# Autodesk Inventor assembly: Frame 1647030135921
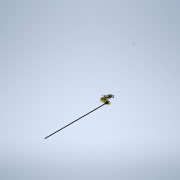
[picture p0: Inventor's stored thumbnail of the model, 180x180]
Saved by Autodesk Inventor 2022.2 (Build 262287000, 287)
## iProperties
_FrameDoc: Frame Assembly
_Version: 25.0.0
Created: 2022-03-11
Part Number: Frame 1647030135921
Document SubType Name: Assembly
Designer: foriw
Mass: 6298.67 g
Surface Area: 9103.39 cm^2
Volume: 2238.81 cm^3
Density: 2.8134 g/cm^3
Author: foriw
## Documents named in this file (31)
- H:\inventor ting\Mekatronik beercart git\Beercart CAD\Workspaces\Workspace\beercart assembly - mekatronik\Frame\Frame 1647030135921.iam
- H:\inventor ting\Mekatronik beercart git\Beercart CAD\Workspaces\Workspace\beercart assembly - mekatronik\Frame\Skeleton 1647030135922.ipt
- H:\inventor ting\Mekatronik beercart git\Beercart CAD\Workspaces\Workspace\beercart assembly - mekatronik\Frame\ISO 12633-2 20x20x2 1647030639616.ipt
- H:\inventor ting\Mekatronik beercart git\Beercart CAD\Workspaces\Workspace\beercart assembly - mekatronik\Frame\ISO 12633-2 20x20x2 1647030639707.ipt
- H:\inventor ting\Mekatronik beercart git\Beercart CAD\Workspaces\Workspace\beercart assembly - mekatronik\Frame\ISO 12633-2 20x20x2 1647606177438.ipt
- H:\inventor ting\Mekatronik beercart git\Beercart CAD\Workspaces\Workspace\BackWheelMountingPlate.ipt
- H:\inventor ting\Mekatronik beercart git\Beercart CAD\Workspaces\Workspace\BackWheelMountingPlate_MIR_MIR.ipt
- H:\inventor ting\Mekatronik beercart git\Beercart CAD\Workspaces\Workspace\bearing housing front.ipt
- H:\inventor ting\Mekatronik beercart git\Beercart CAD\Workspaces\Workspace\beercart assembly - mekatronik\Frame\ISO 12633-2 20x20x2 1648573909221.ipt
- H:\inventor ting\Mekatronik beercart git\Beercart CAD\Workspaces\Workspace\beercart assembly - mekatronik\Frame\ISO 12633-2 20x20x2 1648573975084.ipt
- H:\inventor ting\Mekatronik beercart git\Beercart CAD\Workspaces\Workspace\beercart assembly - mekatronik\Frame\ISO 12633-2 20x20x2 1648627088055.ipt
- H:\inventor ting\Mekatronik beercart git\Beercart CAD\Workspaces\Workspace\beercart assembly - mekatronik\Frame\ISO 12633-2 20x20x2 1648627088175.ipt
- H:\inventor ting\Mekatronik beercart git\Beercart CAD\Workspaces\Workspace\BackWheelMountingPlate_MIR4.ipt
- H:\inventor ting\Mekatronik beercart git\Beercart CAD\Workspaces\Workspace\beercart assembly - mekatronik\Frame\ISO 12633-2 20x20x2 1649085652950.ipt
- H:\inventor ting\Mekatronik beercart git\Beercart CAD\Workspaces\Workspace\beercart assembly - mekatronik\Frame\ISO 12633-2 20x20x2 1649085653040.ipt
- H:\inventor ting\Mekatronik beercart git\Beercart CAD\Workspaces\Workspace\backWheelNoMotor brake mount.ipt
- H:\inventor ting\Mekatronik beercart git\Beercart CAD\Workspaces\Workspace\beercart assembly - mekatronik\Frame\ISO 12633-2 20x20x2 1649154464355.ipt
- H:\inventor ting\Mekatronik beercart git\Beercart CAD\Workspaces\Workspace\BackWheelMotorMountSpacer.ipt
- H:\inventor ting\Mekatronik beercart git\Beercart CAD\Workspaces\Workspace\beercart assembly - mekatronik\Frame\FrontWheelFrameNew.iam
- H:\inventor ting\Mekatronik beercart git\Beercart CAD\Workspaces\Workspace\headset bearing.ipt
- H:\inventor ting\Mekatronik beercart git\Beercart CAD\Workspaces\Workspace\beercart assembly - mekatronik\Frame\ISO 12633-2 20x20x2 1650129877673.ipt
- H:\inventor ting\Mekatronik beercart git\Beercart CAD\Workspaces\Workspace\beercart assembly - mekatronik\Frame\ISO 12633-2 20x20x2 1650129879551.ipt
- H:\inventor ting\Mekatronik beercart git\Beercart CAD\Workspaces\Workspace\beercart assembly - mekatronik\Frame\ISO 12633-2 20x20x2 1650129879650.ipt
- H:\inventor ting\Mekatronik beercart git\Beercart CAD\Workspaces\Workspace\beercart assembly - mekatronik\Frame\ISO 12633-2 20x20x2 1650129879749.ipt
- H:\inventor ting\Mekatronik beercart git\Beercart CAD\Workspaces\Workspace\beercart assembly - mekatronik\Frame\ISO 12633-2 20x20x2 1650134807858.ipt
- H:\inventor ting\Mekatronik beercart git\Beercart CAD\Workspaces\Workspace\bearing housing front_MIR.ipt
- H:\inventor ting\Mekatronik beercart git\Beercart CAD\Libraries\Content Center Files\en-US\ISO 7089\ISO 7089 - 6 - 140 HV(1).ipt
- H:\inventor ting\Mekatronik beercart git\Beercart CAD\Libraries\Content Center Files\en-US\ISO 4762(2)\ISO 4762 - M6 x 16ISO.ipt
- H:\inventor ting\Mekatronik beercart git\Beercart CAD\Workspaces\Workspace\rotating axel.ipt
- H:\inventor ting\Mekatronik beercart git\Beercart CAD\Workspaces\Workspace\beercart assembly - mekatronik\Frame\plan1 .iam
- H:\inventor ting\Mekatronik beercart git\Beercart CAD\Workspaces\Workspace\beercart assembly - mekatronik\Frame\Plan 2 øverste.iam
## Components (36 placed, 26 different names)
1. bearing housing front:1 — Mate:6, Flush:15, Flush:16, Mate:8, Insert:4, Mate:10, Mate:12
2. Reference Skeleton
3. ISO 12633-2 20x20x2 - 250,13:1
4. ISO 12633-2 20x20x2 - 250,13:2
5. ISO 12633-2 20x20x2 - 123,73:2 — Mate:2, Mate:4, Mate:5
6. BackWheelMountingPlate:1 — Flush:6, Rotational:2, Rigid:1
7. BackWheelMountingPlate_MIR_MIR:1
8. ISO 12633-2 20x20x2 - 360,44:1
9. ISO 12633-2 20x20x2 - 105,43:1 — Flush:6, Rotational:2, Rigid:1
10. ISO 12633-2 20x20x2 - 107,97:1 — Flush:9, Flush:11, Flush:12, Flush:13, Rigid:2
11. ISO 12633-2 20x20x2 - 110,27:1
12. BackWheelMountingPlate_MIR4:1 — Flush:9, Rigid:2
13. ISO 12633-2 20x20x2 - 115,53:1 — Flush:14
14. ISO 12633-2 20x20x2 - 113,38:1 — Flush:10
15. backWheelNoMotor brake mount:1 — Flush:10, Flush:14
16. ISO 12633-2 20x20x2 - 105,43:1
17. BackWheelMotorMountSpacer:1 — Flush:11, Flush:12, Flush:13
18. FrontWheelFrameNew:1 [sub-assembly] — Insert:3, Mate:8, Insert:4, Angle:1
19. headset bearing:1 — Insert:3
20. ISO 12633-2 20x20x2 - 76,3:1 — Flush:16
21. ISO 12633-2 20x20x2 - 85,41:1 — Mate:6, Flush:15, Mate:9, Mate:11
22. ISO 12633-2 20x20x2 - 85,41:2 — Flush:17, Mate:7, Mate:13
23. ISO 12633-2 20x20x2 - 76,3:2 — Flush:18, Mate:15
24. ISO 12633-2 20x20x2 - 98,29:1
25. bearing housing front_MIR:1 — Flush:17, Flush:18, Mate:7, Mate:14, Mate:16
26. ISO 7089 6:1 — Mate:9, Mate:10, Insert:5
27. ISO 4762 M6 x 16:1 — Insert:5
28. ISO 7089 6:2 — Mate:11, Mate:12, Insert:6
29. ISO 4762 M6 x 16:2 — Insert:6
30. ISO 7089 6:3 — Mate:13, Mate:14, Insert:7
31. ISO 4762 M6 x 16:3 — Insert:7
32. ISO 7089 6:4 — Mate:15, Mate:16, Insert:8
33. ISO 4762 M6 x 16:4 — Insert:8
34. rotating axel:1 — Flush:19, Angle:1
35. plan1 :1 [sub-assembly]
36. Plan 2 øverste:1 [sub-assembly]
## Relationships (37: Mate 15, Flush 12, Insert 6, WeldJoint 2, RevoluteJoint 1, Angle 1)
- Mate:2: ISO 12633-2 20x20x2 - 123,73:2
- Mate:4: ISO 12633-2 20x20x2 - 123,73:2
- Mate:5: ISO 12633-2 20x20x2 - 123,73:2
- Flush:6: BackWheelMountingPlate:1 ↔ ISO 12633-2 20x20x2 - 105,43:1
- Rotational:2 [RevoluteJoint]: BackWheelMountingPlate:1 ↔ ISO 12633-2 20x20x2 - 105,43:1
- Flush:9: ISO 12633-2 20x20x2 - 107,97:1 ↔ BackWheelMountingPlate_MIR4:1
- Flush:10: ISO 12633-2 20x20x2 - 113,38:1 ↔ backWheelNoMotor brake mount:1
- Rigid:1 [WeldJoint]: BackWheelMountingPlate:1 ↔ ISO 12633-2 20x20x2 - 105,43:1
- Flush:11: ISO 12633-2 20x20x2 - 107,97:1 ↔ BackWheelMotorMountSpacer:1
- Flush:12: ISO 12633-2 20x20x2 - 107,97:1 ↔ BackWheelMotorMountSpacer:1
- Flush:13: ISO 12633-2 20x20x2 - 107,97:1 ↔ BackWheelMotorMountSpacer:1
- Flush:14: ISO 12633-2 20x20x2 - 115,53:1 ↔ backWheelNoMotor brake mount:1
- Insert:3: FrontWheelFrameNew:1 ↔ headset bearing:1
- Rigid:2 [WeldJoint]: ISO 12633-2 20x20x2 - 107,97:1 ↔ BackWheelMountingPlate_MIR4:1
- Mate:6: bearing housing front:1 ↔ ISO 12633-2 20x20x2 - 85,41:1
- Flush:15: bearing housing front:1 ↔ ISO 12633-2 20x20x2 - 85,41:1
- Flush:16: bearing housing front:1 ↔ ISO 12633-2 20x20x2 - 76,3:1
- Flush:17: ISO 12633-2 20x20x2 - 85,41:2 ↔ bearing housing front_MIR:1
- Flush:18: ISO 12633-2 20x20x2 - 76,3:2 ↔ bearing housing front_MIR:1
- Mate:7: ISO 12633-2 20x20x2 - 85,41:2 ↔ bearing housing front_MIR:1
- Mate:8: bearing housing front:1 ↔ FrontWheelFrameNew:1
- Insert:4: bearing housing front:1 ↔ FrontWheelFrameNew:1
- Mate:9: ISO 12633-2 20x20x2 - 85,41:1 ↔ ISO 7089 6:1
- Mate:10: bearing housing front:1 ↔ ISO 7089 6:1
- Insert:5: ISO 7089 6:1 ↔ ISO 4762 M6 x 16:1
- Mate:11: ISO 12633-2 20x20x2 - 85,41:1 ↔ ISO 7089 6:2
- Mate:12: bearing housing front:1 ↔ ISO 7089 6:2
- Insert:6: ISO 7089 6:2 ↔ ISO 4762 M6 x 16:2
- Mate:13: ISO 12633-2 20x20x2 - 85,41:2 ↔ ISO 7089 6:3
- Mate:14: bearing housing front_MIR:1 ↔ ISO 7089 6:3
- Insert:7: ISO 7089 6:3 ↔ ISO 4762 M6 x 16:3
- Mate:15: ISO 12633-2 20x20x2 - 76,3:2 ↔ ISO 7089 6:4
- Mate:16: bearing housing front_MIR:1 ↔ ISO 7089 6:4
- Insert:8: ISO 7089 6:4 ↔ ISO 4762 M6 x 16:4
- [Mate]: bearing housing front:1 ↔ rotating axel:1
- Flush:19: rotating axel:1
- Angle:1 (0 deg): FrontWheelFrameNew:1 ↔ rotating axel:1
## Named parameters: d99_d81 = 0 mm
